# Autodesk Inventor assembly: AnsambluMotor
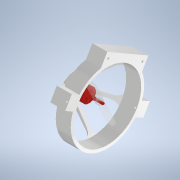
[picture p0: Inventor's stored thumbnail of the model, 180x180]
Saved by Autodesk Inventor 2020.3 (Build 243373000, 373)
## iProperties
Created: 2021-03-16
Part Number: AnsambluMotor
Document SubType Name: Assembly
Designer: alexo
Mass: 130.648 g
Surface Area: 514.455 cm^2
Volume: 124.095 cm^3
Density: 1.05281 g/cm^3
Author: alexo
## iProperties of the stored document BR2212 Body.ipt
Created: 2019-02-23
Part Number: BR2212 Body
Material: Generic
Document SubType Name: Modeling
Designer: alexo
Density: 1 g/cm^3
Appearance: Default
Mass: 13.5478 g
Surface Area: 38.793 cm^2
Volume: 13.5478 cm^3
Author: alexo
Revision Number: ANY
## iProperties of the stored document BR2212 Mount.ipt
Created: 2019-02-23
Part Number: BR2212 Mount
Material: Generic
Document SubType Name: Modeling
Designer: alexo
Density: 1 g/cm^3
Appearance: Default
Mass: 0.920462 g
Surface Area: 13.2147 cm^2
Volume: 0.920462 cm^3
Author: alexo
Revision Number: ANY
## iProperties of the stored document BR2212.iam
Created: 2019-02-23
Part Number: BR2212
Description: STEP AP203
Document SubType Name: Assembly
Designer: alexo
Mass: 14.8751 g
Surface Area: 58.9039 cm^2
Volume: 14.8751 cm^3
Density: 1 g/cm^3
Sending System: SolidWorks 2018
Preprocessor: SwSTEP 2.0
Title: BR2212 Assem..STEP
Revision Number: ANY
## iProperties of the stored document BR2212 Stock.ipt
Created: 2019-02-23
Part Number: BR2212 Stock
Material: Generic
Document SubType Name: Modeling
Designer: alexo
Density: 1 g/cm^3
Appearance: Default
Mass: 0.406919 g
Surface Area: 6.89621 cm^2
Volume: 0.406919 cm^3
Author: alexo
Revision Number: ANY
## Documents named in this file (14)
- C:\Users\alexo\Documents\Inventor\TheArch\R&D\Beta0\Structura\Motor\AnsambluMotor.iam
- C:\Users\alexo\Documents\Inventor\TheArch\R&D\Beta0\Structura\Motor\Prindere.ipt
- **C:\Users\alexo\Documents\Inventor\TheArch\R&D\Beta0\Structura\Motor\AnsambluMotor.iam*LocalDocs*xAaaaaicaAaaaaaaaAaaaqhcjPg*BR2212.iam
- C:\Users\alexo\Documents\Inventor\TheArch\Componente\Elicii\5030\Elice5030.ipt
- **C:\Users\alexo\Documents\Inventor\TheArch\R&D\Beta0\Structura\Motor\AnsambluMotor.iam*LocalDocs*xAaaaabbaAaaaaaaaAaaaazjl2a*BR2212 Body.ipt
- **C:\Users\alexo\Documents\Inventor\TheArch\R&D\Beta0\Structura\Motor\AnsambluMotor.iam*LocalDocs*xAaaaa2caAaaaaaaaAaaaar0aRa*BR2212 Mount.ipt
- **C:\Users\alexo\Documents\Inventor\TheArch\R&D\Beta0\Structura\Motor\AnsambluMotor.iam*LocalDocs*xAaaaqqbaAaaaaaaaAaaaawn32h*BR2212 Stock.ipt
- C:\Users\alexo\Documents\Inventor\TheArch\Componente\Motoare\Motor\BR2212\BR2212.STEP
- C:\Users\alexo\Documents\Inventor\TheArch\R&D\Beta0\Structura\Motor\AnsambluMotor\AIP\FEA\djq0uhnuo.fins
- C:\Users\alexo\Documents\Inventor\TheArch\R&D\Beta0\Structura\Motor\AnsambluMotor\AIP\FEA\djq0uhnuo.fsat
- C:\Users\alexo\Documents\Inventor\TheArch\R&D\Beta0\Structura\Motor\AnsambluMotor\AIP\FEA\djq0uhnuo.ftes
- C:\Users\alexo\Documents\Inventor\TheArch\R&D\Beta0\Structura\Motor\AnsambluMotor\AIP\FEA\djq0uhnuo.fwiz
- C:\Users\alexo\Documents\Inventor\TheArch\R&D\Beta0\Structura\Motor\AnsambluMotor\AIP\FEA\djq0uhnwg.fmsh
- C:\Users\alexo\Documents\Inventor\TheArch\R&D\Beta0\Structura\Motor\AnsambluMotor\AIP\FEA\djq0uhnwh.fres
## Components (3 placed, 3 different names)
1. Prindere:1 — Rigid:1
2. BR2212:1 [sub-assembly] — Rigid:1, Rotational:1
3. Elice5030:1 — Rotational:1
## Relationships (2: WeldJoint 1, RevoluteJoint 1)
- Rigid:1 [WeldJoint]: Prindere:1 ↔ BR2212:1
- Rotational:1 [RevoluteJoint]: BR2212:1 ↔ Elice5030:1
